# Autodesk Inventor assembly: UBG-Rad
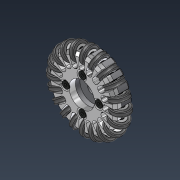
[picture p0: Inventor's stored thumbnail of the model, 180x180]
Saved by Autodesk Inventor 2022.1 (Build 261234020, 234B)
## iProperties
Part Number: UBG-Rad
Material: Generisch
Document SubType Name: Assembly
Designer: rYan
Mass: 53.555 g
Surface Area: 435.52 cm^2
Volume: 34.2485 cm^3
Density: 1.56372 g/cm^3
Author: rYan
## Documents named in this file (6)
- D:\TIGERsGIT\Hardware\mechanik\2020\Inventor\Robot\Drive Train\UBG-Rad.iam
- D:\TIGERsGIT\Hardware\mechanik\2020\Inventor\Robot\Drive Train\Radkasten.ipt
- D:\TIGERsGIT\Hardware\mechanik\2020\Inventor\Robot\Drive Train\MG-Rolle.iam
- D:\TIGERsGIT\Hardware\mechanik\2020\Inventor\Robot\Drive Train\Raddeckel.ipt
- D:\TIGERsGIT\Hardware\mechanik\2020\Inventor\Inhaltscenter\de-DE\ISO 10642(1)\ISO 10642 - M3 x  8.ipt
- D:\TIGERsGIT\Hardware\mechanik\2020\Inventor\Purchased Parts\iC-Haus PX01S 26-360.ipt
## Components (27 placed, 5 different names)
1. Radkasten:1 — Passend:1, Fluchtend:1, Fluchtend:2, Passend:5, Passend:7, Passend:8, Einfügen:1, Passend:9, Passend:11
2. iC-Haus PX01S 26-360:1 — Passend:7, Passend:8
3. Raddeckel:1 — Einfügen:1, Passend:9, Einfügen:2, Einfügen:3, Einfügen:4, Einfügen:5, Passend:10
4. ISO 10642 M3 x  8:1 — Einfügen:2
5. ISO 10642 M3 x  8:2 — Einfügen:4
6. ISO 10642 M3 x  8:3 — Einfügen:5
7. ISO 10642 M3 x  8:4 — Einfügen:3
8. MG-Rolle:1 [sub-assembly] — Passend:2, Winkel:1, Passend:6, Passend:12
9. MG-Rolle:2 [sub-assembly]
10. MG-Rolle:3 [sub-assembly]
11. MG-Rolle:4 [sub-assembly]
12. MG-Rolle:5 [sub-assembly]
13. MG-Rolle:6 [sub-assembly]
14. MG-Rolle:7 [sub-assembly]
15. MG-Rolle:8 [sub-assembly]
16. MG-Rolle:9 [sub-assembly]
17. MG-Rolle:10 [sub-assembly]
18. MG-Rolle:11 [sub-assembly]
19. MG-Rolle:12 [sub-assembly]
20. MG-Rolle:13 [sub-assembly]
21. MG-Rolle:14 [sub-assembly]
22. MG-Rolle:15 [sub-assembly]
23. MG-Rolle:16 [sub-assembly]
24. MG-Rolle:17 [sub-assembly]
25. MG-Rolle:18 [sub-assembly]
26. MG-Rolle:19 [sub-assembly]
27. MG-Rolle:20 [sub-assembly]
## Component patterns: (20 elements, first: MG-Rolle:1)
## Relationships (20: Mate 10, Insert 5, Flush 3, Angle 2)
- Passend:1 [Mate]: Radkasten:1
- Fluchtend:1 [Flush]: Radkasten:1
- Fluchtend:2 [Flush]: Radkasten:1
- Passend:2 [Mate]: MG-Rolle:1
- Winkel:1 [Angle] (0 deg): MG-Rolle:1
- Passend:5 [Mate]: Radkasten:1
- Passend:6 [Mate]: MG-Rolle:1
- Passend:7 [Mate]: Radkasten:1 ↔ iC-Haus PX01S 26-360:1
- Passend:8 [Mate]: Radkasten:1 ↔ iC-Haus PX01S 26-360:1
- Einfügen:1 [Insert]: Radkasten:1 ↔ Raddeckel:1
- Passend:9 [Mate]: Radkasten:1 ↔ Raddeckel:1
- Einfügen:2 [Insert]: Raddeckel:1 ↔ ISO 10642 M3 x  8:1
- Einfügen:3 [Insert]: Raddeckel:1 ↔ ISO 10642 M3 x  8:4
- Einfügen:4 [Insert]: Raddeckel:1 ↔ ISO 10642 M3 x  8:2
- Einfügen:5 [Insert]: Raddeckel:1 ↔ ISO 10642 M3 x  8:3
- Fluchtend:3 [Flush] (31.3 mm)
- Passend:10 [Mate]: Raddeckel:1
- Winkel:2 [Angle] (0 deg)
- Passend:11 [Mate]: Radkasten:1
- Passend:12 [Mate]: MG-Rolle:1
